# Autodesk Inventor assembly: Z assembly
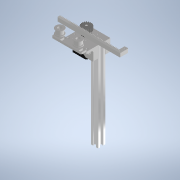
[picture p0: Inventor's stored thumbnail of the model, 180x180]
Saved by Autodesk Inventor 2022 (Build 260153000, 153)
## iProperties
Created: 2022-03-06
Part Number: Z assembly
Document SubType Name: Assembly
Designer: JK
Author: JK
## Documents named in this file (11)
- C:\Users\JK\Documents\Inventor\ScaraNema\SCARA-3DP\Parts\Z axis\Z assembly.iam
- C:\Users\JK\Documents\Inventor\ScaraNema\SCARA-3DP\Parts\Z axis\NEMA14 support.ipt
- C:\Users\JK\Documents\Inventor\ScaraNema\SCARA-3DP\Parts\Z axis\Gear.ipt
- C:\Users\JK\Documents\Inventor\ScaraNema\SCARA-3DP\Parts\Z axis\RackZ.ipt
- C:\Users\JK\Documents\Inventor\ScaraNema\SCARA-3DP\Parts\MOTOR.ipt
- C:\Users\JK\Documents\Inventor\ScaraNema\SCARA-3DP\Parts\V-Slot 20x20\V-Slot 20x20-250.ipt
- C:\Users\JK\Documents\Inventor\ScaraNema\SCARA-3DP\Parts\V-Slot 20x20.ipt
- C:\Users\JK\Documents\Inventor\ScaraNema\SCARA-3DP\Parts\Z axis\Rack support.ipt
- C:\Users\JK\Documents\Inventor\ScaraNema\SCARA-3DP\Parts\Z axis\Bearing.ipt
- C:\Users\JK\Documents\Inventor\ScaraNema\SCARA-3DP\Parts\Z axis\Roller.ipt
- C:\Users\JK\Documents\Inventor\ScaraNema\SCARA-3DP\Parts\Z axis\Separator.ipt
## Components (11 placed, 9 different names)
1. NEMA14 support:1 — Ángulo:2, Coincidencia:3, Ángulo:3, Coincidencia:4, Coincidencia:5, Nivelación:1, Coincidencia:6, Coincidencia:7, Nivelación:5
2. Gear:1 — Coincidencia:1, Coincidencia:2, Coincidencia:3, Nivelación:2
3. RackZ:1 — Ángulo:2, Nivelación:2, Nivelación:3
4. MOTOR:1 — Coincidencia:1, Coincidencia:2, Ángulo:3, Coincidencia:4, Nivelación:3
5. V-Slot 20x20-250:1 — Coincidencia:5, Nivelación:1, Coincidencia:6
6. Rack support:1 — Coincidencia:7, Nivelación:5, Coincidencia:8, Coincidencia:9, Coincidencia:10, Coincidencia:15
7. Bearing:1 — Coincidencia:8, Nivelación:6, Coincidencia:11, Coincidencia:13
8. Bearing:2 — Coincidencia:9, Coincidencia:10, Nivelación:6, Coincidencia:12
9. Roller:1 — Coincidencia:11, Nivelación:7, Coincidencia:13, Coincidencia:14
10. Roller:2 — Coincidencia:12, Nivelación:7
11. Separator:1 — Coincidencia:14, Coincidencia:15
## Relationships (23: Mate 15, Flush 6, Angle 2)
- Ángulo:2 [Angle] (180 deg): NEMA14 support:1 ↔ RackZ:1
- Coincidencia:1 [Mate]: Gear:1 ↔ MOTOR:1
- Coincidencia:2 [Mate] (2.5 mm): Gear:1 ↔ MOTOR:1
- Coincidencia:3 [Mate]: NEMA14 support:1 ↔ Gear:1
- Ángulo:3 [Angle] (0 deg): NEMA14 support:1 ↔ MOTOR:1
- Coincidencia:4 [Mate]: NEMA14 support:1 ↔ MOTOR:1
- Coincidencia:5 [Mate]: NEMA14 support:1 ↔ V-Slot 20x20-250:1
- Nivelación:1 [Flush]: NEMA14 support:1 ↔ V-Slot 20x20-250:1
- Coincidencia:6 [Mate]: NEMA14 support:1 ↔ V-Slot 20x20-250:1
- Nivelación:2 [Flush]: Gear:1 ↔ RackZ:1
- Nivelación:3 [Flush] (-0.5 mm): RackZ:1 ↔ MOTOR:1
- Coincidencia:7 [Mate]: NEMA14 support:1 ↔ Rack support:1
- Nivelación:5 [Flush]: NEMA14 support:1 ↔ Rack support:1
- Coincidencia:8 [Mate]: Rack support:1 ↔ Bearing:1
- Coincidencia:9 [Mate]: Rack support:1 ↔ Bearing:2
- Coincidencia:10 [Mate]: Rack support:1 ↔ Bearing:2
- Nivelación:6 [Flush]: Bearing:1 ↔ Bearing:2
- Coincidencia:11 [Mate]: Bearing:1 ↔ Roller:1
- Coincidencia:12 [Mate]: Bearing:2 ↔ Roller:2
- Nivelación:7 [Flush]: Roller:1 ↔ Roller:2
- Coincidencia:13 [Mate]: Bearing:1 ↔ Roller:1
- Coincidencia:14 [Mate]: Roller:1 ↔ Separator:1
- Coincidencia:15 [Mate]: Rack support:1 ↔ Separator:1
